# Autodesk Inventor assembly: inner_mirrored
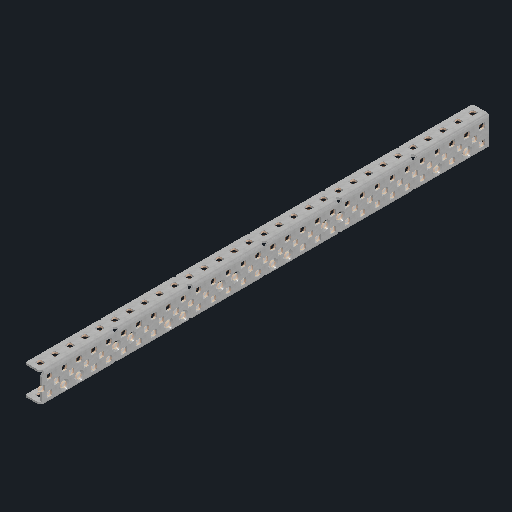
[picture p0: Inventor's stored thumbnail of the model, 512x512]
Saved by Autodesk Inventor 2025 (Build 290162000, 162)
## iProperties
Created: 2024-10-11
Part Number: inner_mirrored
Document SubType Name: Assembly
Designer: Averey Ku
Author: Averey Ku
## Documents named in this file (2)
- D:\vex_robotics_high_stakes\hardware\cad\bots\high_stakes_v2\chassis_v2\drivebay_mirrored\inner_mirrored.iam
- D:\vex_robotics_high_stakes\hardware\cad\bots\high_stakes_v2\chassis_v2\drivebay_mirrored\Alu C 1x2x1x30_mirrored.ipt
## Components (1 placed, 1 different names)
1. Alu C 1x2x1x30_mirrored:1 — Mate:1
## Relationships (1: Mate 1)
- Mate:1: Alu C 1x2x1x30_mirrored:1
